# Autodesk Inventor assembly: ACS770_CurrentSense
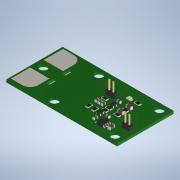
[picture p0: Inventor's stored thumbnail of the model, 180x180]
Saved by Autodesk Inventor 2021 (Build 250183000, 183)
## iProperties
Company: A Company
Created: 2021-05-18
Part Number: ACS770_CurrentSense
Description: KiCad electronic assembly
Document SubType Name: Assembly
Designer: Barksdale
Authority: Unknown
Title: ACS770_CurrentSense.step
Author: An Author
Sending System: KiCad to STEP converter
Preprocessor: Open CASCADE STEP processor 6.9
## Documents named in this file (10)
- C:\Users\Barksdale\Dropbox (MIT)\MPI Group Folder\MPS\MPSV2\4xxx PCB and Filters\42xx Current Sense Circuits\ACS770_CurrentSense.iam
- C:\Users\Barksdale\Dropbox (MIT)\MPI Group Folder\MPS\MPSV2\4xxx PCB and Filters\42xx Current Sense Circuits\SOT-23-5.iam
- C:\Users\Barksdale\Dropbox (MIT)\MPI Group Folder\MPS\MPSV2\4xxx PCB and Filters\42xx Current Sense Circuits\R_1206_3216Metric.iam
- C:\Users\Barksdale\Dropbox (MIT)\MPI Group Folder\MPS\MPSV2\4xxx PCB and Filters\42xx Current Sense Circuits\C_0805_2012Metric.iam
- C:\Users\Barksdale\Dropbox (MIT)\MPI Group Folder\MPS\MPSV2\4xxx PCB and Filters\42xx Current Sense Circuits\LED_1206_3216Metric.iam
- C:\Users\Barksdale\Dropbox (MIT)\MPI Group Folder\MPS\MPSV2\4xxx PCB and Filters\42xx Current Sense Circuits\C_1206_3216Metric.iam
- C:\Users\Barksdale\Dropbox (MIT)\MPI Group Folder\MPS\MPSV2\4xxx PCB and Filters\42xx Current Sense Circuits\SOIC-8_3.9x4.9mm_P1.27mm.iam
- C:\Users\Barksdale\Dropbox (MIT)\MPI Group Folder\MPS\MPSV2\4xxx PCB and Filters\42xx Current Sense Circuits\PinHeader_1x02_P2.54mm_Vertical.iam
- C:\Users\Barksdale\Dropbox (MIT)\MPI Group Folder\MPS\MPSV2\4xxx PCB and Filters\42xx Current Sense Circuits\COMPOUND.ipt
- C:\Users\Barksdale\Dropbox (MIT)\MPI Group Folder\MPS\MPSV2\4xxx PCB and Filters\42xx Current Sense Circuits\4201_ACS770_Solder_Pads_MPSv2_v1.ipt
## Components (26 placed, 25 different names)
1. 2 [sub-assembly]
2. 4 [sub-assembly]
3. 5 [sub-assembly]
4. 6 [sub-assembly]
5. 7 [sub-assembly]
6. 9 [sub-assembly]
7. 10 [sub-assembly]
8. 11 [sub-assembly]
9. 13 [sub-assembly]
10. 15 [sub-assembly]
11. 17 [sub-assembly]
12. 18 [sub-assembly]
13. 19 [sub-assembly]
14. 20 [sub-assembly]
15. 21 [sub-assembly]
16. 23 [sub-assembly]
17. 24 [sub-assembly]
18. 25 [sub-assembly]
19. 26 [sub-assembly]
20. 27 [sub-assembly]
21. 28 [sub-assembly]
22. 29 [sub-assembly]
23. 30 [sub-assembly]
24. 31 — Mate:1, Mate:2, Angle:1, Angle:2
25. 4201_ACS770_Solder_Pads_MPSv2_v1:1 — Mate:2, Angle:1
26. 4201_ACS770_Solder_Pads_MPSv2_v1:2 — Mate:1, Angle:2
## Relationships (4: Mate 2, Angle 2)
- Mate:1: 31 ↔ 4201_ACS770_Solder_Pads_MPSv2_v1:2
- Mate:2: 31 ↔ 4201_ACS770_Solder_Pads_MPSv2_v1:1
- Angle:1 (0 deg): 31 ↔ 4201_ACS770_Solder_Pads_MPSv2_v1:1
- Angle:2 (0 deg): 31 ↔ 4201_ACS770_Solder_Pads_MPSv2_v1:2
